# Autodesk Inventor assembly: 0837 solenoid
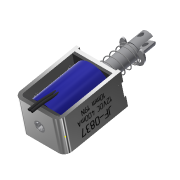
[picture p0: Inventor's stored thumbnail of the model, 180x180]
Saved by Autodesk Inventor 2018.1 (Build 221171000, 171)
## iProperties
Created: 2019-06-27
Part Number: 0837 solenoid
Material: Типовые
Document SubType Name: Assembly
Designer: Boss
Mass: 46.6308 g
Surface Area: 145.209 cm^2
Volume: 15.6816 cm^3
Density: 2.97361 g/cm^3
Author: Boss
## Documents named in this file (9)
- D:\Gujenov-LAB\3D модели изделий\Электрика и электромеханика\silenoids\0837\0837 solenoid.iam
- D:\Gujenov-LAB\3D модели изделий\Электрика и электромеханика\silenoids\0837\base.ipt
- D:\Gujenov-LAB\3D модели изделий\Электрика и электромеханика\silenoids\0837\cover.ipt
- D:\Gujenov-LAB\3D модели изделий\Электрика и электромеханика\silenoids\0837\frame.ipt
- D:\Gujenov-LAB\3D модели изделий\Электрика и электромеханика\silenoids\0837\coil.ipt
- D:\Gujenov-LAB\3D модели изделий\Электрика и электромеханика\silenoids\0837\nut.ipt
- D:\Gujenov-LAB\3D модели изделий\Электрика и электромеханика\silenoids\0837\kern.ipt
- C:\Users\Boss\Documents\Inventor\Content Center Files\R2018\ru-RU\DIN 6799\DIN 6799 - 7 8.ipt
- D:\Gujenov-LAB\3D модели изделий\Электрика и электромеханика\silenoids\0837\0837 solenoid\Мастер проектирования\Пружина сжатия2.iam
## Components (8 placed, 8 different names)
1. base:1 — Совмещение:1, Совмещение:2, Совмещение:4, Совмещение:6, Вставка:1, Совмещение:9, Совмещение:10
2. cover:1 — Совмещение:1, Совмещение:2, Совмещение:5, Заподлицо:2, Совмещение:10
3. frame:1 — Совмещение:4, Совмещение:5, Совмещение:6, Заподлицо:1, Жесткий:2, Совмещение:7
4. coil:1 — Заподлицо:1, Жесткий:2
5. nut:1 — Вставка:1
6. kern:1 — Совмещение:7, Вставка:2, Совмещение:8
7. DIN 6799 7:1 — Вставка:2
8. Пружина сжатия:1 [sub-assembly] — Совмещение:8, Заподлицо:2
## Relationships (14: Mate 9, Flush 2, Insert 2, WeldJoint 1)
- Совмещение:1 [Mate]: base:1 ↔ cover:1
- Совмещение:2 [Mate]: base:1 ↔ cover:1
- Совмещение:4 [Mate]: base:1 ↔ frame:1
- Совмещение:5 [Mate]: cover:1 ↔ frame:1
- Совмещение:6 [Mate]: base:1 ↔ frame:1
- Заподлицо:1 [Flush]: frame:1 ↔ coil:1
- Вставка:1 [Insert]: base:1 ↔ nut:1
- Жесткий:2 [WeldJoint]: frame:1 ↔ coil:1
- Совмещение:7 [Mate]: frame:1 ↔ kern:1
- Вставка:2 [Insert]: kern:1 ↔ DIN 6799 7:1
- Совмещение:8 [Mate]: kern:1 ↔ Пружина сжатия:1
- Заподлицо:2 [Flush]: cover:1 ↔ Пружина сжатия:1
- Совмещение:9 [Mate]: base:1
- Совмещение:10 [Mate]: base:1 ↔ cover:1
